# Autodesk Inventor assembly: 3t2000
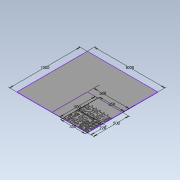
[picture p0: Inventor's stored thumbnail of the model, 180x180]
Saved by Autodesk Inventor 2020.3 (Build 243373000, 373)
## iProperties
Created: 2020-05-22
Part Number: 3t2000
Document SubType Name: Assembly
Designer: aoyama
Author: aoyama
## Documents named in this file (13)
- C:\Users\aoyam\Desktop\SRDC_local\Inventor\二年機\Geminiβ\3t2000.iam
- C:\Users\aoyam\Desktop\SRDC_local\Inventor\二年機\AL板サイズ測定板.ipt
- C:\Users\aoyam\Desktop\SRDC_local\Inventor\二年機\Geminiβ\脚\中間ユニット\中間フレーム内側.ipt
- C:\Users\aoyam\Desktop\SRDC_local\Inventor\二年機\Geminiβ\脚\中間ユニット\脚中間フレーム外側.ipt
- C:\Users\aoyam\Desktop\SRDC_local\Inventor\二年機\Geminiβ\汎用部品\ｍ2歯数17ギアd3.99.ipt
- C:\Users\aoyam\Desktop\SRDC_local\Inventor\二年機\Geminiβ\汎用部品\ｍ2歯数14ギアd10.ipt
- C:\Users\aoyam\Desktop\SRDC_local\Inventor\二年機\Geminiβ\腕\アームフレーム改二.ipt
- C:\Users\aoyam\Desktop\SRDC_local\Inventor\二年機\Geminiβ\腕\モーターマウント改.ipt
- C:\Users\aoyam\Desktop\SRDC_local\Inventor\二年機\Geminiβ\腕\アーム揺動節抑え.ipt
- C:\Users\aoyam\Desktop\SRDC_local\Inventor\二年機\Geminiβ\腕\アーム底板.ipt
- C:\Users\aoyam\Desktop\SRDC_local\Inventor\二年機\Geminiβ\エンドミルモデル.ipt
- C:\Users\aoyam\Desktop\SRDC_local\Inventor\二年機\Geminiβ\脚\脚ギアトレイン2.ipt
- C:\Users\aoyam\Desktop\SRDC_local\Inventor\二年機\Geminiβ\脚\ネジクランク\揺動節.ipt
## Components (42 placed, 12 different names)
1. AL板サイズ測定板:1 — メイト:1, メイト:2, メイト:3, メイト:4, メイト:5, メイト:6, メイト:7, メイト:8, メイト:9, メイト:10, メイト:11, メイト:12, メイト:13, メイト:14, メイト:15, メイト:18, メイト:19, メイト:20, メイト:21, メイト:22, メイト:23, メイト:24, メイト:25, メイト:26, メイト:27, メイト:28, メイト:29, メイト:30, メイト:31, メイト:32, メイト:33, メイト:34, メイト:35, メイト:36, メイト:37, メイト:38, メイト:39, メイト:40
2. 中間フレーム内側:1 — メイト:1
3. 中間フレーム内側:2 — メイト:2
4. 脚中間フレーム外側:1 — メイト:3
5. 脚中間フレーム外側:2 — メイト:4
6. ｍ2歯数17ギアd3.99:1 — メイト:5
7. ｍ2歯数17ギアd3.99:2 — メイト:6
8. ｍ2歯数17ギアd3.99:3 — メイト:7
9. ｍ2歯数17ギアd3.99:4 — メイト:8
10. ｍ2歯数14ギアd10:1 — フラッシュ:1
11. ｍ2歯数14ギアd10:2 — フラッシュ:1, フラッシュ:2, メイト:9
12. ｍ2歯数14ギアd10:3 — フラッシュ:2, フラッシュ:3
13. ｍ2歯数14ギアd10:4 — フラッシュ:3
14. アームフレーム改二:1 — メイト:10, 角度:1
15. アームフレーム改二:2 — メイト:11, 角度:1
16. モーターマウント改:1 — メイト:12
17. モーターマウント改:2 — メイト:13
18. アーム揺動節抑え:1 — メイト:14
19. アーム揺動節抑え:2 — メイト:15
20. アーム底板:1 — メイト:18, 角度:2
21. アーム底板:2 — メイト:20, 角度:2
22. エンドミルモデル:1 — メイト:19
23. 脚ギアトレイン2:1 — メイト:23
24. 脚ギアトレイン2:2 — メイト:24
25. 脚ギアトレイン2:3 — メイト:21
26. 脚ギアトレイン2:4 — メイト:22
27. 揺動節:1 — メイト:33
28. 揺動節:2 — メイト:34
29. 揺動節:3 — メイト:32
30. 揺動節:4 — メイト:31
31. 揺動節:5 — メイト:30
32. 揺動節:6 — メイト:35
33. 揺動節:7 — メイト:36
34. 揺動節:8 — メイト:37
35. 揺動節:9 — メイト:29
36. 揺動節:10 — メイト:38
37. 揺動節:11 — メイト:25
38. 揺動節:12 — メイト:26
39. 揺動節:13 — メイト:27
40. 揺動節:14 — メイト:28
41. 揺動節:15 — メイト:40
42. 揺動節:16 — メイト:39
## Relationships (43: Mate 38, Flush 3, Angle 2)
- メイト:1 [Mate]: AL板サイズ測定板:1 ↔ 中間フレーム内側:1
- メイト:2 [Mate]: AL板サイズ測定板:1 ↔ 中間フレーム内側:2
- メイト:3 [Mate]: AL板サイズ測定板:1 ↔ 脚中間フレーム外側:1
- メイト:4 [Mate]: AL板サイズ測定板:1 ↔ 脚中間フレーム外側:2
- メイト:5 [Mate]: AL板サイズ測定板:1 ↔ ｍ2歯数17ギアd3.99:1
- メイト:6 [Mate]: AL板サイズ測定板:1 ↔ ｍ2歯数17ギアd3.99:2
- メイト:7 [Mate]: AL板サイズ測定板:1 ↔ ｍ2歯数17ギアd3.99:3
- メイト:8 [Mate]: AL板サイズ測定板:1 ↔ ｍ2歯数17ギアd3.99:4
- フラッシュ:1 [Flush]: ｍ2歯数14ギアd10:1 ↔ ｍ2歯数14ギアd10:2
- フラッシュ:2 [Flush]: ｍ2歯数14ギアd10:2 ↔ ｍ2歯数14ギアd10:3
- フラッシュ:3 [Flush]: ｍ2歯数14ギアd10:3 ↔ ｍ2歯数14ギアd10:4
- メイト:9 [Mate]: AL板サイズ測定板:1 ↔ ｍ2歯数14ギアd10:2
- メイト:10 [Mate]: AL板サイズ測定板:1 ↔ アームフレーム改二:1
- メイト:11 [Mate]: AL板サイズ測定板:1 ↔ アームフレーム改二:2
- 角度:1 [Angle] (180 deg): アームフレーム改二:1 ↔ アームフレーム改二:2
- メイト:12 [Mate]: AL板サイズ測定板:1 ↔ モーターマウント改:1
- メイト:13 [Mate]: AL板サイズ測定板:1 ↔ モーターマウント改:2
- メイト:14 [Mate]: AL板サイズ測定板:1 ↔ アーム揺動節抑え:1
- メイト:15 [Mate]: AL板サイズ測定板:1 ↔ アーム揺動節抑え:2
- メイト:18 [Mate]: AL板サイズ測定板:1 ↔ アーム底板:1
- メイト:19 [Mate]: AL板サイズ測定板:1 ↔ エンドミルモデル:1
- メイト:20 [Mate]: AL板サイズ測定板:1 ↔ アーム底板:2
- 角度:2 [Angle] (180 deg): アーム底板:1 ↔ アーム底板:2
- メイト:21 [Mate]: AL板サイズ測定板:1 ↔ 脚ギアトレイン2:3
- メイト:22 [Mate]: AL板サイズ測定板:1 ↔ 脚ギアトレイン2:4
- メイト:23 [Mate]: AL板サイズ測定板:1 ↔ 脚ギアトレイン2:1
- メイト:24 [Mate]: AL板サイズ測定板:1 ↔ 脚ギアトレイン2:2
- メイト:25 [Mate]: AL板サイズ測定板:1 ↔ 揺動節:11
- メイト:26 [Mate]: AL板サイズ測定板:1 ↔ 揺動節:12
- メイト:27 [Mate]: AL板サイズ測定板:1 ↔ 揺動節:13
- メイト:28 [Mate]: AL板サイズ測定板:1 ↔ 揺動節:14
- メイト:29 [Mate]: AL板サイズ測定板:1 ↔ 揺動節:9
- メイト:30 [Mate]: AL板サイズ測定板:1 ↔ 揺動節:5
- メイト:31 [Mate]: AL板サイズ測定板:1 ↔ 揺動節:4
- メイト:32 [Mate]: AL板サイズ測定板:1 ↔ 揺動節:3
- メイト:33 [Mate]: AL板サイズ測定板:1 ↔ 揺動節:1
- メイト:34 [Mate]: AL板サイズ測定板:1 ↔ 揺動節:2
- メイト:35 [Mate]: AL板サイズ測定板:1 ↔ 揺動節:6
- メイト:36 [Mate]: AL板サイズ測定板:1 ↔ 揺動節:7
- メイト:37 [Mate]: AL板サイズ測定板:1 ↔ 揺動節:8
- メイト:38 [Mate]: AL板サイズ測定板:1 ↔ 揺動節:10
- メイト:39 [Mate]: AL板サイズ測定板:1 ↔ 揺動節:16
- メイト:40 [Mate]: AL板サイズ測定板:1 ↔ 揺動節:15
